# Autodesk Inventor assembly: 1103 Lift -Top Tier
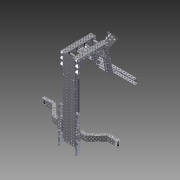
[picture p0: Inventor's stored thumbnail of the model, 180x180]
Saved by Autodesk Inventor 2012 (Build 160160000, 160)
## iProperties
Created: 2011-08-16
Part Number: 1103 Lift -Top Tier
Document SubType Name: Assembly
Designer: Dakota.Bayer
Author: Dakota.Bayer
## Documents named in this file (32)
- C:\Users\Wade\Documents\1103 Robot - CAD Assembly\1103 Lift -Top Tier.iam
- C:\Users\Wade\Documents\1103 Robot - CAD Assembly\5 x 30.ipt
- C:\Users\Wade\Documents\1103 Robot - CAD Assembly\1103 laddercustom1.ipt
- C:\Users\Wade\Documents\1103 Robot - CAD Assembly\2 x 12 c chan.ipt
- C:\Users\Wade\Documents\1103 Robot - CAD Assembly\1 x 10.ipt
- C:\Users\Wade\Documents\1103 Robot - CAD Assembly\Thin Black Spacer.ipt
- C:\Users\Wade\Documents\1103 Robot - CAD Assembly\2 x 20.ipt
- C:\Users\Wade\Documents\1103 Robot - CAD Assembly\2 x 41103 custom.ipt
- C:\Users\Wade\Documents\1103 Robot - CAD Assembly\2 x 15 custom!!!.iam
- C:\Users\Wade\Documents\1103 Robot - CAD Assembly\VEX-HINGE-PIN.ipt
- C:\Users\Wade\Documents\1103 Robot - CAD Assembly\VEX-HINGE-1 RevA.ipt
- C:\Users\Wade\Documents\24C VEX CAD Files\Standoffs & Couplers\Standoff 0.50''.ipt
- C:\Users\Wade\Documents\24C VEX CAD Files\Screws & Nuts\Screw 8-32 x 0.250''-Silver.ipt
- C:\Users\Wade\Documents\24C VEX CAD Files\Washers & Spacers\Spacer (Nylon), 0.375''.ipt
- C:\Users\Wade\Documents\24C VEX CAD Files\Screws & Nuts\Screw 8-32 x 0.750''-Silver.ipt
- C:\Users\Wade\Documents\24C VEX CAD Files\Screws & Nuts\Screw 8-32 x 0.375''-Silver.ipt
- C:\Users\Wade\Documents\24C VEX CAD Files\Screws & Nuts\Nut 8-32 Nylock.ipt
- C:\Users\Wade\Documents\24C VEX CAD Files\Washers & Spacers\Spacer (Nylon), 0.250''.ipt
- C:\Users\Wade\Documents\24C VEX CAD Files\Screws & Nuts\Screw 8-32 x 0.500''-Silver.ipt
- C:\Users\Wade\Documents\24C VEX CAD Files\Standoffs & Couplers\Standoff 0.75''.ipt
- C:\Users\Wade\Documents\24C VEX CAD Files\Standoffs & Couplers\Standoff 1.50''.ipt
- C:\Users\Wade\Documents\24C VEX CAD Files\Metal Other\Linear Slide Assembly-Parts\Linear Slide-Inner.ipt
- C:\Users\Wade\Documents\24C VEX CAD Files\Washers & Spacers\Spacer (Nylon), 0.4375''.ipt
- C:\Users\Wade\Documents\24C VEX CAD Files\Standoffs & Couplers\Standoff 3.00''.ipt
- C:\Users\Wade\Documents\24C VEX CAD Files\Standoffs & Couplers\Standoff 1.00''.ipt
- C:\Users\Wade\Documents\1103 Robot - CAD Assembly\.375'' Screw & Nylock Nut (Custom).iam
- C:\Users\Wade\Documents\1103 Robot - CAD Assembly\.375'' Screw & Nylock Nut.iam
- C:\Users\Wade\Documents\24C VEX CAD Files\Screws & Nuts\Screw 8-32 x 0.875''-Silver.ipt
- C:\Users\Wade\Documents\24C VEX CAD Files\Chain & Tank Tread\High Strength Chain Link.ipt
- C:\Users\Wade\Documents\1103 Robot - CAD Assembly\Ladder Mech.iam
- C:\Users\Wade\Documents\24C VEX CAD Files\Screws & Nuts\Screw 8-32 x 0.625''-Silver.ipt
- C:\Users\Wade\Documents\24C VEX CAD Files\Screws & Nuts\Screw 8-32 x 1.250''-Silver.ipt
## Components (161 placed, 31 different names)
1. 5 x 30:1 — Flush:33, Flush:34, Mate:310, Flush:35, Flush:36, Mate:328, Mate:693, Flush:43, Flush:44, Mate:757, Flush:53, Flush:54, Mate:774, Mate:775, Mate:776, Mate:778, Mate:779, Mate:780, Mate:823, Mate:825
2. Linear Slide-Inner:1
3. Standoff 0.50'':1
4. Screw 8-32 x 0.250''-Silver:1
5. Screw 8-32 x 0.250''-Silver:2
6. Screw 8-32 x 0.250''-Silver:3
7. Screw 8-32 x 0.250''-Silver:4
8. Standoff 0.50'':2
9. Screw 8-32 x 0.250''-Silver:5
10. Standoff 0.50'':3
11. Linear Slide-Inner:2
12. Screw 8-32 x 0.250''-Silver:6
13. Screw 8-32 x 0.250''-Silver:7
14. Screw 8-32 x 0.250''-Silver:8
15. Standoff 0.50'':4
16. Screw 8-32 x 0.250''-Silver:9 — Mate:804, Mate:805
17. 1103 laddercustom1:1 — Flush:33, Flush:34, Mate:474, Mate:818, Mate:819, Mate:821
18. Nut 8-32 Nylock:1
19. Nut 8-32 Nylock:2
20. Nut 8-32 Nylock:3
21. Screw 8-32 x 0.750''-Silver:4
22. Screw 8-32 x 0.750''-Silver:6 — Mate:818
23. Screw 8-32 x 0.750''-Silver:5 — Mate:820
24. 2 x 12 c chan:1 — Mate:310, Mate:459, Mate:474, Mate:500, Mate:505, Mate:512, Mate:515, Mate:837, Tangent:458, Tangent:459, Mate:840, Tangent:460, Tangent:461, Mate:841
25. Screw 8-32 x 0.375''-Silver:1
26. Screw 8-32 x 0.375''-Silver:2
27. Nut 8-32 Nylock:4
28. Nut 8-32 Nylock:5
29. 1103 laddercustom1:2 — Flush:35, Flush:36, Mate:484
30. Screw 8-32 x 0.750''-Silver:1 — Mate:822
31. Nut 8-32 Nylock:6
32. Screw 8-32 x 0.750''-Silver:2 — Mate:824
33. Nut 8-32 Nylock:7
34. 2 x 12 c chan:2 — Mate:328, Mate:460, Mate:484, Mate:503, Mate:507, Mate:509, Mate:518, Tangent:450, Tangent:451, Mate:835, Tangent:454, Tangent:455, Mate:838, Tangent:456, Tangent:457, Mate:839, Angle:1
35. Nut 8-32 Nylock:8
36. Screw 8-32 x 0.750''-Silver:3
37. Screw 8-32 x 0.375''-Silver:3
38. Nut 8-32 Nylock:9
39. Screw 8-32 x 0.375''-Silver:4
40. Nut 8-32 Nylock:10
41. 2 x 12 c chan:3 — Flush:37, Flush:38, Mate:460, Mate:525, Mate:794, Mate:795, Mate:796, Mate:797, Mate:798, Mate:799, Mate:828, Mate:829, Tangent:462, Tangent:463, Mate:876, Mate:877, Mate:885
42. 2 x 12 c chan:4 — Flush:37, Flush:38, Mate:459, Mate:788, Mate:789, Mate:790, Mate:791, Mate:792, Mate:793, Mate:814, Mate:815, Mate:875, Mate:881, Mate:884
43. 1 x 10:1 — Mate:843, Mate:872, Mate:875
44. 1 x 10:2 — Mate:525, Tangent:452, Tangent:453, Mate:845, Tangent:468, Tangent:469
45. Standoff 1.00'':1
46. Screw 8-32 x 0.375''-Silver:5
47. Screw 8-32 x 0.375''-Silver:6
48. Screw 8-32 x 0.375''-Silver:7
49. Screw 8-32 x 0.375''-Silver:8
50. Standoff 1.00'':2
51. Screw 8-32 x 0.375''-Silver:9
52. Screw 8-32 x 0.375''-Silver:10
53. Standoff 1.00'':3
54. Screw 8-32 x 0.375''-Silver:11
55. Screw 8-32 x 0.375''-Silver:12
56. Standoff 1.00'':4
57. Spacer (Nylon), 0.375'':1
58. Spacer (Nylon), 0.4375'':1 — Mate:819
59. Spacer (Nylon), 0.375'':6
60. Thin Black Spacer:1 — Mate:500
61. Thin Black Spacer:2 — Mate:503
62. Thin Black Spacer:3 — Mate:505
63. Thin Black Spacer:4 — Mate:507
64. Thin Black Spacer:5 — Mate:512
65. Thin Black Spacer:6 — Mate:509
66. Thin Black Spacer:7 — Mate:518
67. Thin Black Spacer:8 — Mate:515
68. Screw 8-32 x 0.375''-Silver:13
69. Screw 8-32 x 0.375''-Silver:14
70. Standoff 1.50'':1
71. Screw 8-32 x 0.375''-Silver:15
72. Screw 8-32 x 0.375''-Silver:16
73. Standoff 1.50'':2
74. Screw 8-32 x 0.375''-Silver:17
75. Screw 8-32 x 0.375''-Silver:18
76. Standoff 1.50'':3
77. Screw 8-32 x 0.375''-Silver:19
78. Screw 8-32 x 0.375''-Silver:20
79. Standoff 1.50'':4
80. Screw 8-32 x 0.375''-Silver:21
81. Screw 8-32 x 0.375''-Silver:22
82. Standoff 1.50'':5
83. Standoff 3.00'':1
84. Spacer (Nylon), 0.250'':1 — Mate:873
85. Spacer (Nylon), 0.250'':2
86. Screw 8-32 x 0.500''-Silver:1
87. Screw 8-32 x 0.500''-Silver:2 — Mate:872
88. Screw 8-32 x 0.500''-Silver:3
89. Screw 8-32 x 0.500''-Silver:4
90. Spacer (Nylon), 0.250'':3 — Mate:874
91. Standoff 3.00'':2 — Mate:873, Mate:874
92. Spacer (Nylon), 0.250'':4
93. 2 x 20:1 — Mate:800, Mate:801, Mate:802, Mate:803, Mate:805, Mate:807, Mate:810, Mate:811
94. Screw 8-32 x 0.625''-Silver:2 — Mate:879, Mate:889, Mate:890
95. Screw 8-32 x 0.625''-Silver:1 — Mate:880, Mate:886, Mate:891
96. Standoff 0.50'':5 — Mate:765, Mate:768, Mate:854
97. Standoff 0.50'':6 — Mate:760, Mate:763, Mate:846, Mate:905
98. Standoff 0.50'':7 — Mate:766, Mate:767, Mate:856
99. Standoff 0.50'':8 — Mate:761, Mate:762, Mate:848
100. Standoff 0.50'':9 — Mate:773, Mate:777, Mate:778, Mate:779, Mate:780, Mate:860
101. Standoff 0.50'':10 — Mate:770, Mate:771, Mate:772, Mate:774, Mate:775, Mate:776, Mate:858
102. 2 x 41103 custom:1 — Mate:693, Flush:43, Flush:44, Flush:66, Flush:67, Mate:904
103. 2 x 15 custom!!!:1 [sub-assembly] — Flush:66, Flush:67, Mate:894, Mate:896, Mate:897, Mate:904
104. Standoff 0.50'':11 — Mate:783, Mate:784, Mate:850
105. Standoff 0.50'':12 — Mate:782, Mate:785, Mate:852
106. 2 x 15 custom!!!:2 [sub-assembly] — Flush:64, Flush:65, Mate:898, Mate:900, Mate:901, Mate:903
107. 2 x 41103 custom:2 — Mate:757, Flush:53, Flush:54, Flush:64, Flush:65, Mate:903
108. VEX-HINGE-PIN:1 — Mate:759, Flush:60
109. VEX-HINGE-1 RevA:1 — Mate:759, Flush:60, Mate:760, Mate:761, Mate:762, Mate:763, Mate:847, Mate:849, Mate:905
110. VEX-HINGE-1 RevA:2 — Mate:764, Flush:61, Mate:765, Mate:766, Mate:767, Mate:768, Mate:855, Mate:857
111. VEX-HINGE-PIN:2 — Mate:764, Flush:61
112. VEX-HINGE-1 RevA:3 — Mate:769, Flush:62, Mate:770, Mate:771, Mate:772, Mate:773, Mate:777, Mate:859, Mate:861
113. VEX-HINGE-PIN:3 — Mate:769, Flush:62
114. VEX-HINGE-1 RevA:4 — Flush:63, Mate:781, Mate:782, Mate:783, Mate:784, Mate:785, Mate:851, Mate:853
115. VEX-HINGE-PIN:4 — Flush:63, Mate:781
116. Standoff 0.75'':1 — Mate:788, Mate:789, Mate:790, Mate:804, Mate:813
117. Standoff 0.75'':2 — Mate:794, Mate:795, Mate:796, Mate:809, Mate:826
118. Standoff 0.75'':3 — Mate:797, Mate:798, Mate:799, Mate:800, Mate:801, Mate:802, Mate:808, Mate:827
119. Standoff 0.75'':4 — Mate:791, Mate:792, Mate:793, Mate:803, Mate:806, Mate:812
120. Screw 8-32 x 0.250''-Silver:10 — Mate:806, Mate:807
121. Screw 8-32 x 0.250''-Silver:11 — Mate:808, Mate:811
122. Screw 8-32 x 0.250''-Silver:12 — Mate:809, Mate:810
123. Screw 8-32 x 0.250''-Silver:13 — Mate:812, Mate:814
124. Screw 8-32 x 0.250''-Silver:14 — Mate:813, Mate:815
125. Spacer (Nylon), 0.4375'':2 — Mate:820, Mate:821
126. Spacer (Nylon), 0.4375'':3 — Mate:824, Mate:825
127. Spacer (Nylon), 0.4375'':4 — Mate:822, Mate:823
128. Screw 8-32 x 0.250''-Silver:15 — Mate:827, Mate:829
129. Screw 8-32 x 0.250''-Silver:16 — Mate:826, Mate:828
130. .375'' Screw & Nylock Nut (Custom):1 [sub-assembly] — Tangent:450, Tangent:451, Mate:835, Tangent:452, Tangent:453, Mate:836
131. .375'' Screw & Nylock Nut (Custom):2 [sub-assembly] — Mate:836, Mate:837
132. .375'' Screw & Nylock Nut:1 [sub-assembly] — Tangent:454, Tangent:455, Mate:838, Tangent:462, Tangent:463
133. .375'' Screw & Nylock Nut:2 [sub-assembly] — Tangent:460, Tangent:461, Mate:841
134. .375'' Screw & Nylock Nut:3 [sub-assembly] — Tangent:458, Tangent:459, Mate:840
135. .375'' Screw & Nylock Nut:4 [sub-assembly] — Tangent:456, Tangent:457, Mate:839
136. .375'' Screw & Nylock Nut:5 [sub-assembly] — Mate:843, Mate:878
137. .375'' Screw & Nylock Nut:6 [sub-assembly] — Mate:845, Mate:876, Mate:877, Tangent:468, Tangent:469, Mate:878
138. Screw 8-32 x 0.250''-Silver:17 — Mate:848, Mate:849
139. Screw 8-32 x 0.250''-Silver:18 — Mate:850, Mate:851
140. Screw 8-32 x 0.250''-Silver:19 — Mate:852, Mate:853
141. Screw 8-32 x 0.250''-Silver:20 — Mate:846, Mate:847
142. Screw 8-32 x 0.250''-Silver:21 — Mate:854, Mate:855
143. Screw 8-32 x 0.250''-Silver:22 — Mate:856, Mate:857
144. Screw 8-32 x 0.250''-Silver:23 — Mate:858, Mate:859
145. Screw 8-32 x 0.250''-Silver:24 — Mate:860, Mate:861
146. Screw 8-32 x 0.875''-Silver:1 — Mate:865, Tangent:466, Tangent:467
147. Nut 8-32 Nylock:21 — Mate:865, Mate:869
148. Spacer (Nylon), 0.375'':7 — Mate:868, Mate:869, Mate:870
149. High Strength Chain Link:1 — Mate:868, Tangent:466, Mate:870, Tangent:467, Mate:871, Flush:68
150. High Strength Chain Link:2 — Mate:871, Flush:68
151. Ladder Mech:1 [sub-assembly] — Mate:879, Mate:880, Mate:881, Mate:882, Mate:883, Angle:1
152. Screw 8-32 x 0.750''-Silver:7 — Mate:882, Mate:885, Mate:887, Mate:892
153. Screw 8-32 x 0.750''-Silver:8 — Mate:883, Mate:884, Mate:888, Mate:893
154. Nut 8-32 Nylock:22 — Mate:888, Mate:893
155. Nut 8-32 Nylock:23 — Mate:889, Mate:890
156. Nut 8-32 Nylock:24 — Mate:887, Mate:892
157. Nut 8-32 Nylock:25 — Mate:886, Mate:891
158. Nut 8-32 Nylock:26 — Mate:895, Mate:896
159. Screw 8-32 x 1.250''-Silver:1 — Mate:894, Mate:895, Mate:897
160. Nut 8-32 Nylock:27 — Mate:900, Mate:902
161. Screw 8-32 x 1.250''-Silver:2 — Mate:898, Mate:901, Mate:902
## Relationships (415: Mate 274, Tangent 120, Flush 20, Angle 1)
- [Flush]: 5 x 30:1 ↔ Linear Slide-Inner:1
- [Mate]: 5 x 30:1 ↔ Standoff 0.50'':1
- [Mate]: 5 x 30:1 ↔ Screw 8-32 x 0.250''-Silver:1
- [Mate]: Linear Slide-Inner:1 ↔ Screw 8-32 x 0.250''-Silver:2
- [Mate]: Standoff 0.50'':1 ↔ Screw 8-32 x 0.250''-Silver:1
- [Mate]: Standoff 0.50'':1 ↔ Screw 8-32 x 0.250''-Silver:2
- [Mate]: Linear Slide-Inner:1 ↔ Standoff 0.50'':1
- [Mate]: Linear Slide-Inner:1 ↔ Screw 8-32 x 0.250''-Silver:4
- [Tangent] (0.2286 mm): Linear Slide-Inner:1 ↔ Screw 8-32 x 0.250''-Silver:4
- [Tangent] (0.2286 mm): Linear Slide-Inner:1 ↔ Screw 8-32 x 0.250''-Silver:4
- [Mate]: Linear Slide-Inner:1 ↔ Standoff 0.50'':2
- [Mate]: Screw 8-32 x 0.250''-Silver:4 ↔ Standoff 0.50'':2
- [Mate]: 5 x 30:1 ↔ Standoff 0.50'':2
- [Mate]: 5 x 30:1 ↔ Screw 8-32 x 0.250''-Silver:3
- [Mate]: 5 x 30:1 ↔ Screw 8-32 x 0.250''-Silver:5
- [Mate]: 5 x 30:1 ↔ Standoff 0.50'':3
- [Mate]: Screw 8-32 x 0.250''-Silver:5 ↔ Standoff 0.50'':3
- [Mate]: Standoff 0.50'':3 ↔ Linear Slide-Inner:2
- [Mate]: Linear Slide-Inner:2 ↔ Screw 8-32 x 0.250''-Silver:6
- [Tangent] (0.2286 mm): Linear Slide-Inner:2 ↔ Screw 8-32 x 0.250''-Silver:6
- [Tangent] (0.2286 mm): Linear Slide-Inner:2 ↔ Screw 8-32 x 0.250''-Silver:6
- [Mate]: Standoff 0.50'':3 ↔ Screw 8-32 x 0.250''-Silver:6
- [Mate]: 5 x 30:1 ↔ Screw 8-32 x 0.250''-Silver:7
- [Tangent] (0.2286 mm): 5 x 30:1 ↔ Screw 8-32 x 0.250''-Silver:7
- [Tangent] (0.2286 mm): 5 x 30:1 ↔ Screw 8-32 x 0.250''-Silver:7
- [Mate]: Linear Slide-Inner:2 ↔ Screw 8-32 x 0.250''-Silver:8
- [Mate]: 5 x 30:1 ↔ Standoff 0.50'':4
- [Mate]: Linear Slide-Inner:2 ↔ Standoff 0.50'':4
- [Mate]: Screw 8-32 x 0.250''-Silver:8 ↔ Standoff 0.50'':4
- [Mate]: Screw 8-32 x 0.250''-Silver:7 ↔ Standoff 0.50'':4
- Flush:33: 5 x 30:1 ↔ 1103 laddercustom1:1
- Flush:34: 5 x 30:1 ↔ 1103 laddercustom1:1
- [Mate]: 5 x 30:1 ↔ Nut 8-32 Nylock:1
- [Mate]: 5 x 30:1 ↔ Nut 8-32 Nylock:2
- [Mate]: 5 x 30:1 ↔ Nut 8-32 Nylock:3
- [Tangent] (0.2286 mm): 1103 laddercustom1:1 ↔ Screw 8-32 x 0.750''-Silver:6
- [Tangent] (0.2286 mm): 1103 laddercustom1:1 ↔ Screw 8-32 x 0.750''-Silver:6
- [Mate]: Nut 8-32 Nylock:3 ↔ Screw 8-32 x 0.750''-Silver:6
- [Tangent] (0.2286 mm): 1103 laddercustom1:1 ↔ Screw 8-32 x 0.750''-Silver:5
- [Tangent] (0.2286 mm): 1103 laddercustom1:1 ↔ Screw 8-32 x 0.750''-Silver:5
- [Mate]: Nut 8-32 Nylock:2 ↔ Screw 8-32 x 0.750''-Silver:5
- [Tangent] (0.2286 mm): 1103 laddercustom1:1 ↔ Screw 8-32 x 0.750''-Silver:4
- [Tangent] (0.2286 mm): 1103 laddercustom1:1 ↔ Screw 8-32 x 0.750''-Silver:4
- [Tangent] (0.2286 mm): Screw 8-32 x 0.750''-Silver:4 ↔ 2 x 12 c chan:1
- Mate:310: 5 x 30:1 ↔ 2 x 12 c chan:1
- [Tangent] (0.2286 mm): Screw 8-32 x 0.750''-Silver:4 ↔ 2 x 12 c chan:1
- [Tangent] (0.2286 mm): 1103 laddercustom1:1 ↔ Screw 8-32 x 0.375''-Silver:1
- [Tangent] (0.2286 mm): 1103 laddercustom1:1 ↔ Screw 8-32 x 0.375''-Silver:1
- [Tangent] (0.2286 mm): 1103 laddercustom1:1 ↔ Screw 8-32 x 0.375''-Silver:2
- [Tangent] (0.2286 mm): 1103 laddercustom1:1 ↔ Screw 8-32 x 0.375''-Silver:2
- [Mate]: Screw 8-32 x 0.375''-Silver:2 ↔ Nut 8-32 Nylock:5
- [Mate]: Screw 8-32 x 0.375''-Silver:1 ↔ Nut 8-32 Nylock:4
- Flush:35: 5 x 30:1 ↔ 1103 laddercustom1:2
- Flush:36: 5 x 30:1 ↔ 1103 laddercustom1:2
- [Tangent] (0.2286 mm): 1103 laddercustom1:2 ↔ Screw 8-32 x 0.750''-Silver:1
- [Tangent] (0.2286 mm): 1103 laddercustom1:2 ↔ Screw 8-32 x 0.750''-Silver:1
- [Mate]: 5 x 30:1 ↔ Nut 8-32 Nylock:6
- [Mate]: Screw 8-32 x 0.750''-Silver:1 ↔ Nut 8-32 Nylock:6
- [Tangent] (0.2286 mm): 1103 laddercustom1:2 ↔ Screw 8-32 x 0.750''-Silver:2
- [Tangent] (0.2286 mm): 1103 laddercustom1:2 ↔ Screw 8-32 x 0.750''-Silver:2
- [Mate]: 5 x 30:1 ↔ Nut 8-32 Nylock:7
- [Mate]: Screw 8-32 x 0.750''-Silver:2 ↔ Nut 8-32 Nylock:7
- Mate:328: 5 x 30:1 ↔ 2 x 12 c chan:2
- [Tangent] (0.2286 mm): 1103 laddercustom1:2 ↔ Screw 8-32 x 0.750''-Silver:3
- [Tangent] (0.2286 mm): 1103 laddercustom1:2 ↔ Screw 8-32 x 0.750''-Silver:3
- [Tangent] (0.2286 mm): 5 x 30:1 ↔ Screw 8-32 x 0.750''-Silver:3
- [Tangent] (0.2286 mm): 5 x 30:1 ↔ Screw 8-32 x 0.750''-Silver:3
- [Mate]: 5 x 30:1 ↔ Nut 8-32 Nylock:8
- [Mate]: Nut 8-32 Nylock:8 ↔ Screw 8-32 x 0.750''-Silver:3
- [Tangent] (0.2286 mm): 1103 laddercustom1:2 ↔ Screw 8-32 x 0.375''-Silver:3
- [Tangent] (0.2286 mm): 1103 laddercustom1:2 ↔ Screw 8-32 x 0.375''-Silver:3
- [Mate]: Screw 8-32 x 0.375''-Silver:3 ↔ Nut 8-32 Nylock:9
- [Tangent] (0.2286 mm): 1103 laddercustom1:2 ↔ Screw 8-32 x 0.375''-Silver:4
- [Tangent] (0.2286 mm): 1103 laddercustom1:2 ↔ Screw 8-32 x 0.375''-Silver:4
- [Mate]: Screw 8-32 x 0.375''-Silver:4 ↔ Nut 8-32 Nylock:10
- [Tangent] (0.2286 mm): 2 x 12 c chan:2 ↔ Screw 8-32 x 0.750''-Silver:3
- [Mate]: 2 x 12 c chan:1 ↔ Screw 8-32 x 0.375''-Silver:6
- [Tangent] (0.2286 mm): 2 x 12 c chan:1 ↔ Screw 8-32 x 0.375''-Silver:6
- [Tangent] (0.2286 mm): 2 x 12 c chan:1 ↔ Screw 8-32 x 0.375''-Silver:6
- [Mate]: 2 x 12 c chan:2 ↔ Screw 8-32 x 0.375''-Silver:5
- [Tangent] (0.2286 mm): 2 x 12 c chan:2 ↔ Screw 8-32 x 0.375''-Silver:5
- [Tangent] (0.2286 mm): 2 x 12 c chan:2 ↔ Screw 8-32 x 0.375''-Silver:5
- [Mate]: Standoff 1.00'':1 ↔ Screw 8-32 x 0.375''-Silver:5
- [Mate]: 2 x 12 c chan:1 ↔ Screw 8-32 x 0.375''-Silver:7
- [Tangent] (0.2286 mm): 2 x 12 c chan:1 ↔ Screw 8-32 x 0.375''-Silver:7
- [Tangent] (0.2286 mm): 2 x 12 c chan:1 ↔ Screw 8-32 x 0.375''-Silver:7
- [Mate]: 2 x 12 c chan:2 ↔ Screw 8-32 x 0.375''-Silver:8
- [Tangent] (0.2286 mm): 2 x 12 c chan:2 ↔ Screw 8-32 x 0.375''-Silver:8
- [Tangent] (0.2286 mm): 2 x 12 c chan:2 ↔ Screw 8-32 x 0.375''-Silver:8
- [Mate]: Screw 8-32 x 0.375''-Silver:8 ↔ Standoff 1.00'':2
- [Mate]: 2 x 12 c chan:1 ↔ Screw 8-32 x 0.375''-Silver:9
- [Tangent] (0.2286 mm): 2 x 12 c chan:1 ↔ Screw 8-32 x 0.375''-Silver:9
- [Tangent] (0.2286 mm): 2 x 12 c chan:1 ↔ Screw 8-32 x 0.375''-Silver:9
- [Mate]: 2 x 12 c chan:2 ↔ Screw 8-32 x 0.375''-Silver:10
- [Tangent] (0.2286 mm): 2 x 12 c chan:2 ↔ Screw 8-32 x 0.375''-Silver:10
- [Tangent] (0.2286 mm): 2 x 12 c chan:2 ↔ Screw 8-32 x 0.375''-Silver:10
- [Mate]: Screw 8-32 x 0.375''-Silver:9 ↔ Standoff 1.00'':3
- [Mate]: 2 x 12 c chan:2 ↔ Screw 8-32 x 0.375''-Silver:12
- [Tangent] (0.2286 mm): 2 x 12 c chan:2 ↔ Screw 8-32 x 0.375''-Silver:12
- [Tangent] (0.2286 mm): 2 x 12 c chan:2 ↔ Screw 8-32 x 0.375''-Silver:12
- [Mate]: 2 x 12 c chan:1 ↔ Screw 8-32 x 0.375''-Silver:11
- [Tangent] (0.2286 mm): 2 x 12 c chan:1 ↔ Screw 8-32 x 0.375''-Silver:11
- [Tangent] (0.2286 mm): 2 x 12 c chan:1 ↔ Screw 8-32 x 0.375''-Silver:11
- [Mate]: Screw 8-32 x 0.375''-Silver:12 ↔ Standoff 1.00'':4
- Flush:37: 2 x 12 c chan:3 ↔ 2 x 12 c chan:4
- Flush:38: 2 x 12 c chan:3 ↔ 2 x 12 c chan:4
- Mate:459: 2 x 12 c chan:1 ↔ 2 x 12 c chan:4
- Mate:460: 2 x 12 c chan:2 ↔ 2 x 12 c chan:3
- [Mate]: 5 x 30:1 ↔ Spacer (Nylon), 0.375'':1
- [Mate]: Screw 8-32 x 0.750''-Silver:4 ↔ Spacer (Nylon), 0.375'':1
- Mate:474: 1103 laddercustom1:1 ↔ 2 x 12 c chan:1
- [Mate]: 2 x 12 c chan:1 ↔ Spacer (Nylon), 0.375'':1
- [Mate]: 1103 laddercustom1:1 ↔ Screw 8-32 x 0.750''-Silver:4
- [Mate]: 1103 laddercustom1:1 ↔ Screw 8-32 x 0.375''-Silver:1
- [Mate]: 1103 laddercustom1:1 ↔ Screw 8-32 x 0.375''-Silver:2
- [Mate]: 1103 laddercustom1:1 ↔ Screw 8-32 x 0.750''-Silver:5
- [Mate]: Screw 8-32 x 0.750''-Silver:6 ↔ Spacer (Nylon), 0.4375'':1
- Mate:484: 1103 laddercustom1:2 ↔ 2 x 12 c chan:2
- [Mate]: 1103 laddercustom1:2 ↔ Screw 8-32 x 0.750''-Silver:3
- [Mate]: 5 x 30:1 ↔ Spacer (Nylon), 0.375'':6
- [Mate]: 2 x 12 c chan:2 ↔ Spacer (Nylon), 0.375'':6
- [Mate]: Screw 8-32 x 0.750''-Silver:3 ↔ Spacer (Nylon), 0.375'':6
- [Mate]: 1103 laddercustom1:2 ↔ Screw 8-32 x 0.750''-Silver:2
- [Mate]: 1103 laddercustom1:2 ↔ Screw 8-32 x 0.750''-Silver:1
- [Mate]: 2 x 12 c chan:2 ↔ Nut 8-32 Nylock:10
- [Mate]: 2 x 12 c chan:2 ↔ Nut 8-32 Nylock:9
- [Mate]: Nut 8-32 Nylock:1 ↔ Screw 8-32 x 0.750''-Silver:4
- Mate:500: 2 x 12 c chan:1 ↔ Thin Black Spacer:1
- [Mate]: Screw 8-32 x 0.375''-Silver:11 ↔ Thin Black Spacer:1
- [Mate]: Standoff 1.00'':4 ↔ Thin Black Spacer:1
- Mate:503: 2 x 12 c chan:2 ↔ Thin Black Spacer:2
- [Mate]: Screw 8-32 x 0.375''-Silver:12 ↔ Thin Black Spacer:2
- Mate:505: 2 x 12 c chan:1 ↔ Thin Black Spacer:3
- [Mate]: Screw 8-32 x 0.375''-Silver:9 ↔ Thin Black Spacer:3
- Mate:507: 2 x 12 c chan:2 ↔ Thin Black Spacer:4
- [Mate]: Screw 8-32 x 0.375''-Silver:10 ↔ Thin Black Spacer:4
- Mate:509: 2 x 12 c chan:2 ↔ Thin Black Spacer:6
- [Mate]: Screw 8-32 x 0.375''-Silver:8 ↔ Thin Black Spacer:6
- [Mate]: Standoff 1.00'':3 ↔ Thin Black Spacer:3
- Mate:512: 2 x 12 c chan:1 ↔ Thin Black Spacer:5
- [Mate]: Screw 8-32 x 0.375''-Silver:7 ↔ Thin Black Spacer:5
- [Mate]: Standoff 1.00'':2 ↔ Thin Black Spacer:5
- Mate:515: 2 x 12 c chan:1 ↔ Thin Black Spacer:8
- [Mate]: Screw 8-32 x 0.375''-Silver:6 ↔ Thin Black Spacer:8
- [Mate]: Standoff 1.00'':1 ↔ Thin Black Spacer:8
- Mate:518: 2 x 12 c chan:2 ↔ Thin Black Spacer:7
- [Mate]: Screw 8-32 x 0.375''-Silver:5 ↔ Thin Black Spacer:7
- Mate:525: 2 x 12 c chan:3 ↔ 1 x 10:2
- [Tangent] (0.2286 mm): 2 x 12 c chan:4 ↔ Screw 8-32 x 0.375''-Silver:13
- [Tangent] (0.2286 mm): 2 x 12 c chan:4 ↔ Screw 8-32 x 0.375''-Silver:13
- [Mate]: 2 x 12 c chan:3 ↔ Screw 8-32 x 0.375''-Silver:14
- [Tangent] (0.2286 mm): 2 x 12 c chan:3 ↔ Screw 8-32 x 0.375''-Silver:14
- [Tangent] (0.2286 mm): 2 x 12 c chan:3 ↔ Screw 8-32 x 0.375''-Silver:14
- [Mate]: 2 x 12 c chan:4 ↔ Screw 8-32 x 0.375''-Silver:13
- [Mate]: 2 x 12 c chan:3 ↔ Standoff 1.50'':1
- [Mate]: Screw 8-32 x 0.375''-Silver:14 ↔ Standoff 1.50'':1
- [Mate]: 2 x 12 c chan:3 ↔ Screw 8-32 x 0.375''-Silver:17
- [Tangent] (0.2286 mm): 2 x 12 c chan:3 ↔ Screw 8-32 x 0.375''-Silver:17
- [Tangent] (0.2286 mm): 2 x 12 c chan:3 ↔ Screw 8-32 x 0.375''-Silver:17
- [Mate]: 2 x 12 c chan:4 ↔ Screw 8-32 x 0.375''-Silver:15
- [Tangent] (0.2286 mm): 2 x 12 c chan:4 ↔ Screw 8-32 x 0.375''-Silver:15
- [Tangent] (0.2286 mm): 2 x 12 c chan:4 ↔ Screw 8-32 x 0.375''-Silver:15
- [Mate]: 2 x 12 c chan:3 ↔ Standoff 1.50'':2
- [Mate]: Standoff 1.50'':2 ↔ Screw 8-32 x 0.375''-Silver:17
- [Mate]: 2 x 12 c chan:4 ↔ Screw 8-32 x 0.375''-Silver:18
- [Tangent] (0.2286 mm): 2 x 12 c chan:4 ↔ Screw 8-32 x 0.375''-Silver:18
- [Tangent] (0.2286 mm): 2 x 12 c chan:4 ↔ Screw 8-32 x 0.375''-Silver:18
- [Mate]: 2 x 12 c chan:3 ↔ Screw 8-32 x 0.375''-Silver:16
- [Tangent] (0.2286 mm): 2 x 12 c chan:3 ↔ Screw 8-32 x 0.375''-Silver:16
- [Tangent] (0.2286 mm): 2 x 12 c chan:3 ↔ Screw 8-32 x 0.375''-Silver:16
- [Mate]: 2 x 12 c chan:3 ↔ Standoff 1.50'':3
- [Mate]: Screw 8-32 x 0.375''-Silver:16 ↔ Standoff 1.50'':3
- [Mate]: 2 x 12 c chan:4 ↔ Screw 8-32 x 0.375''-Silver:19
- [Tangent] (0.2286 mm): 2 x 12 c chan:4 ↔ Screw 8-32 x 0.375''-Silver:19
- [Tangent] (0.2286 mm): 2 x 12 c chan:4 ↔ Screw 8-32 x 0.375''-Silver:19
- [Mate]: 2 x 12 c chan:3 ↔ Screw 8-32 x 0.375''-Silver:20
- [Tangent] (0.2286 mm): 2 x 12 c chan:3 ↔ Screw 8-32 x 0.375''-Silver:20
- [Tangent] (0.2286 mm): 2 x 12 c chan:3 ↔ Screw 8-32 x 0.375''-Silver:20
- [Mate]: 2 x 12 c chan:3 ↔ Standoff 1.50'':4
- [Mate]: Screw 8-32 x 0.375''-Silver:20 ↔ Standoff 1.50'':4
- [Mate]: 2 x 12 c chan:4 ↔ Screw 8-32 x 0.375''-Silver:21
- [Tangent] (0.2286 mm): 2 x 12 c chan:4 ↔ Screw 8-32 x 0.375''-Silver:21
- [Tangent] (0.2286 mm): 2 x 12 c chan:4 ↔ Screw 8-32 x 0.375''-Silver:21
- [Mate]: 2 x 12 c chan:3 ↔ Screw 8-32 x 0.375''-Silver:22
- [Tangent] (0.2286 mm): 2 x 12 c chan:3 ↔ Screw 8-32 x 0.375''-Silver:22
- [Tangent] (0.2286 mm): 2 x 12 c chan:3 ↔ Screw 8-32 x 0.375''-Silver:22
- [Mate]: 2 x 12 c chan:3 ↔ Standoff 1.50'':5
- [Mate]: Screw 8-32 x 0.375''-Silver:22 ↔ Standoff 1.50'':5
- [Mate]: 1 x 10:2 ↔ Screw 8-32 x 0.500''-Silver:1
- [Tangent] (0.2286 mm): 1 x 10:2 ↔ Screw 8-32 x 0.500''-Silver:1
- [Tangent] (0.2286 mm): 1 x 10:2 ↔ Screw 8-32 x 0.500''-Silver:1
- [Tangent] (0.2286 mm): 1 x 10:1 ↔ Screw 8-32 x 0.500''-Silver:2
- [Tangent] (0.2286 mm): 1 x 10:1 ↔ Screw 8-32 x 0.500''-Silver:2
- [Mate]: Spacer (Nylon), 0.250'':1 ↔ Screw 8-32 x 0.500''-Silver:2
- [Mate]: 1 x 10:2 ↔ Spacer (Nylon), 0.250'':2
- [Mate]: Spacer (Nylon), 0.250'':2 ↔ Screw 8-32 x 0.500''-Silver:1
- [Mate]: Standoff 3.00'':1 ↔ Spacer (Nylon), 0.250'':2
- [Mate]: Standoff 3.00'':1 ↔ Spacer (Nylon), 0.250'':1
- [Mate]: 1 x 10:2 ↔ Screw 8-32 x 0.500''-Silver:3
- [Tangent] (0.2286 mm): 1 x 10:2 ↔ Screw 8-32 x 0.500''-Silver:3
- [Tangent] (0.2286 mm): 1 x 10:2 ↔ Screw 8-32 x 0.500''-Silver:3
- [Mate]: 1 x 10:1 ↔ Screw 8-32 x 0.500''-Silver:4
- [Tangent] (0.2286 mm): 1 x 10:1 ↔ Screw 8-32 x 0.500''-Silver:4
- [Tangent] (0.2286 mm): 1 x 10:1 ↔ Screw 8-32 x 0.500''-Silver:4
- [Mate]: Screw 8-32 x 0.500''-Silver:4 ↔ Spacer (Nylon), 0.250'':3
- [Mate]: 1 x 10:2 ↔ Spacer (Nylon), 0.250'':4
- [Mate]: Screw 8-32 x 0.500''-Silver:3 ↔ Spacer (Nylon), 0.250'':4
- [Mate]: Standoff 3.00'':2 ↔ Spacer (Nylon), 0.250'':4
- [Mate]: Screw 8-32 x 0.500''-Silver:3 ↔ Standoff 3.00'':2
- [Mate]: 2 x 12 c chan:4 ↔ Screw 8-32 x 0.625''-Silver:2
- [Tangent] (0.2286 mm): 2 x 12 c chan:4 ↔ Screw 8-32 x 0.625''-Silver:2
- [Tangent] (0.2286 mm): 2 x 12 c chan:4 ↔ Screw 8-32 x 0.625''-Silver:2
- [Mate]: 2 x 12 c chan:3 ↔ Screw 8-32 x 0.625''-Silver:1
- [Tangent] (0.2286 mm): 2 x 12 c chan:3 ↔ Screw 8-32 x 0.625''-Silver:1
- [Tangent] (0.2286 mm): 2 x 12 c chan:3 ↔ Screw 8-32 x 0.625''-Silver:1
- [Tangent] (0.2286 mm): Linear Slide-Inner:2 ↔ Screw 8-32 x 0.250''-Silver:8
- [Tangent] (0.2286 mm): Linear Slide-Inner:2 ↔ Screw 8-32 x 0.250''-Silver:8
- [Tangent] (0.2286 mm): 5 x 30:1 ↔ Screw 8-32 x 0.250''-Silver:5
- [Tangent] (0.2286 mm): 5 x 30:1 ↔ Screw 8-32 x 0.250''-Silver:5
- [Tangent] (0.2286 mm): Linear Slide-Inner:1 ↔ Screw 8-32 x 0.250''-Silver:2
- [Tangent] (0.2286 mm): Linear Slide-Inner:1 ↔ Screw 8-32 x 0.250''-Silver:2
- [Tangent] (0.2286 mm): 5 x 30:1 ↔ Screw 8-32 x 0.250''-Silver:1
- [Tangent] (0.2286 mm): 5 x 30:1 ↔ Screw 8-32 x 0.250''-Silver:1
- [Tangent] (0.2286 mm): 5 x 30:1 ↔ Screw 8-32 x 0.250''-Silver:3
- [Tangent] (0.2286 mm): 5 x 30:1 ↔ Screw 8-32 x 0.250''-Silver:3
- [Mate]: 5 x 30:1 ↔ Standoff 0.50'':5
- [Tangent] (0.2286 mm): 5 x 30:1 ↔ Standoff 0.50'':5
- [Tangent] (0.2286 mm): 5 x 30:1 ↔ Standoff 0.50'':5
- [Mate]: 5 x 30:1 ↔ Standoff 0.50'':6
- [Tangent] (0.2159 mm): 5 x 30:1 ↔ Standoff 0.50'':6
- [Tangent] (0.2159 mm): 5 x 30:1 ↔ Standoff 0.50'':6
- [Mate]: 5 x 30:1 ↔ Standoff 0.50'':7
- [Tangent] (0.2286 mm): 5 x 30:1 ↔ Standoff 0.50'':5
- [Tangent] (0.2286 mm): 5 x 30:1 ↔ Standoff 0.50'':7
- [Tangent] (0.2286 mm): 5 x 30:1 ↔ Standoff 0.50'':7
- [Mate]: 5 x 30:1 ↔ Standoff 0.50'':8
- [Tangent] (0.2159 mm): 5 x 30:1 ↔ Standoff 0.50'':8
- [Tangent] (0.2159 mm): 5 x 30:1 ↔ Standoff 0.50'':8
- Mate:693: 5 x 30:1 ↔ 2 x 41103 custom:1
- Flush:43: 5 x 30:1 ↔ 2 x 41103 custom:1
- Flush:44: 5 x 30:1 ↔ 2 x 41103 custom:1
- [Mate]: 5 x 30:1 ↔ Standoff 0.50'':11
- [Mate]: 5 x 30:1 ↔ Standoff 0.50'':12
- [Tangent] (0.2286 mm): 5 x 30:1 ↔ Standoff 0.50'':12
- [Tangent] (0.2286 mm): 5 x 30:1 ↔ Standoff 0.50'':12
- [Tangent] (0.2286 mm): 5 x 30:1 ↔ Standoff 0.50'':11
- [Tangent] (0.2286 mm): 5 x 30:1 ↔ Standoff 0.50'':11
- Mate:757: 5 x 30:1 ↔ 2 x 41103 custom:2
- Flush:53: 5 x 30:1 ↔ 2 x 41103 custom:2
- Flush:54: 5 x 30:1 ↔ 2 x 41103 custom:2
- Mate:759: VEX-HINGE-PIN:1 ↔ VEX-HINGE-1 RevA:1
- Flush:60: VEX-HINGE-PIN:1 ↔ VEX-HINGE-1 RevA:1
- Mate:760: Standoff 0.50'':6 ↔ VEX-HINGE-1 RevA:1
- Mate:761 (2.3114 mm): Standoff 0.50'':8 ↔ VEX-HINGE-1 RevA:1
- Mate:762 (2.3114 mm): Standoff 0.50'':8 ↔ VEX-HINGE-1 RevA:1
- Mate:763 (2.3114 mm): Standoff 0.50'':6 ↔ VEX-HINGE-1 RevA:1
- Mate:764: VEX-HINGE-1 RevA:2 ↔ VEX-HINGE-PIN:2
- Flush:61: VEX-HINGE-1 RevA:2 ↔ VEX-HINGE-PIN:2
- Mate:765: Standoff 0.50'':5 ↔ VEX-HINGE-1 RevA:2
- Mate:766 (2.3114 mm): Standoff 0.50'':7 ↔ VEX-HINGE-1 RevA:2
- Mate:767 (2.3114 mm): Standoff 0.50'':7 ↔ VEX-HINGE-1 RevA:2
- Mate:768 (2.3114 mm): Standoff 0.50'':5 ↔ VEX-HINGE-1 RevA:2
- Mate:769: VEX-HINGE-1 RevA:3 ↔ VEX-HINGE-PIN:3
- Flush:62: VEX-HINGE-1 RevA:3 ↔ VEX-HINGE-PIN:3
- Mate:770: Standoff 0.50'':10 ↔ VEX-HINGE-1 RevA:3
- Mate:771 (2.3114 mm): Standoff 0.50'':10 ↔ VEX-HINGE-1 RevA:3
- Mate:772 (2.3114 mm): Standoff 0.50'':10 ↔ VEX-HINGE-1 RevA:3
- Mate:773 (2.3114 mm): Standoff 0.50'':9 ↔ VEX-HINGE-1 RevA:3
- Mate:774: 5 x 30:1 ↔ Standoff 0.50'':10
- Mate:775 (2.3114 mm): 5 x 30:1 ↔ Standoff 0.50'':10
- Mate:776 (2.3114 mm): 5 x 30:1 ↔ Standoff 0.50'':10
- Mate:777 (2.3114 mm): Standoff 0.50'':9 ↔ VEX-HINGE-1 RevA:3
- Mate:778 (2.3114 mm): 5 x 30:1 ↔ Standoff 0.50'':9
- Mate:779: 5 x 30:1 ↔ Standoff 0.50'':9
- Mate:780 (2.3114 mm): 5 x 30:1 ↔ Standoff 0.50'':9
- Flush:63: VEX-HINGE-1 RevA:4 ↔ VEX-HINGE-PIN:4
- Mate:781: VEX-HINGE-1 RevA:4 ↔ VEX-HINGE-PIN:4
- Mate:782: Standoff 0.50'':12 ↔ VEX-HINGE-1 RevA:4
- Mate:783 (2.3114 mm): Standoff 0.50'':11 ↔ VEX-HINGE-1 RevA:4
- Mate:784 (2.3114 mm): Standoff 0.50'':11 ↔ VEX-HINGE-1 RevA:4
- Mate:785 (2.3114 mm): Standoff 0.50'':12 ↔ VEX-HINGE-1 RevA:4
- Flush:64: 2 x 15 custom!!!:2 ↔ 2 x 41103 custom:2
- Flush:65: 2 x 15 custom!!!:2 ↔ 2 x 41103 custom:2
- Flush:66: 2 x 41103 custom:1 ↔ 2 x 15 custom!!!:1
- Flush:67: 2 x 41103 custom:1 ↔ 2 x 15 custom!!!:1
- Mate:788 (2.3114 mm): 2 x 12 c chan:4 ↔ Standoff 0.75'':1
- Mate:789 (2.3114 mm): 2 x 12 c chan:4 ↔ Standoff 0.75'':1
- Mate:790: 2 x 12 c chan:4 ↔ Standoff 0.75'':1
- Mate:791 (2.3114 mm): 2 x 12 c chan:4 ↔ Standoff 0.75'':4
- Mate:792 (2.3114 mm): 2 x 12 c chan:4 ↔ Standoff 0.75'':4
- Mate:793: 2 x 12 c chan:4 ↔ Standoff 0.75'':4
- Mate:794 (2.3114 mm): 2 x 12 c chan:3 ↔ Standoff 0.75'':2
- Mate:795 (2.3114 mm): 2 x 12 c chan:3 ↔ Standoff 0.75'':2
- Mate:796: 2 x 12 c chan:3 ↔ Standoff 0.75'':2
- Mate:797 (2.3114 mm): 2 x 12 c chan:3 ↔ Standoff 0.75'':3
- Mate:798 (2.3114 mm): 2 x 12 c chan:3 ↔ Standoff 0.75'':3
- Mate:799: 2 x 12 c chan:3 ↔ Standoff 0.75'':3
- Mate:800: 2 x 20:1 ↔ Standoff 0.75'':3
- Mate:801 (1.524 mm): 2 x 20:1 ↔ Standoff 0.75'':3
- Mate:802 (2.3114 mm): 2 x 20:1 ↔ Standoff 0.75'':3
- Mate:803 (2.3114 mm): 2 x 20:1 ↔ Standoff 0.75'':4
- Mate:804: Screw 8-32 x 0.250''-Silver:9 ↔ Standoff 0.75'':1
- Mate:805: Screw 8-32 x 0.250''-Silver:9 ↔ 2 x 20:1
- Mate:806: Standoff 0.75'':4 ↔ Screw 8-32 x 0.250''-Silver:10
- Mate:807: 2 x 20:1 ↔ Screw 8-32 x 0.250''-Silver:10
- Mate:808: Standoff 0.75'':3 ↔ Screw 8-32 x 0.250''-Silver:11
- Mate:809: Standoff 0.75'':2 ↔ Screw 8-32 x 0.250''-Silver:12
- Mate:810: 2 x 20:1 ↔ Screw 8-32 x 0.250''-Silver:12
- Mate:811: 2 x 20:1 ↔ Screw 8-32 x 0.250''-Silver:11
- Mate:812: Standoff 0.75'':4 ↔ Screw 8-32 x 0.250''-Silver:13
- Mate:813: Standoff 0.75'':1 ↔ Screw 8-32 x 0.250''-Silver:14
- Mate:814: 2 x 12 c chan:4 ↔ Screw 8-32 x 0.250''-Silver:13
- Mate:815: 2 x 12 c chan:4 ↔ Screw 8-32 x 0.250''-Silver:14
- Mate:818: 1103 laddercustom1:1 ↔ Screw 8-32 x 0.750''-Silver:6
- Mate:819: 1103 laddercustom1:1 ↔ Spacer (Nylon), 0.4375'':1
- Mate:820: Screw 8-32 x 0.750''-Silver:5 ↔ Spacer (Nylon), 0.4375'':2
- Mate:821: 1103 laddercustom1:1 ↔ Spacer (Nylon), 0.4375'':2
- Mate:822: Screw 8-32 x 0.750''-Silver:1 ↔ Spacer (Nylon), 0.4375'':4
- Mate:823: 5 x 30:1 ↔ Spacer (Nylon), 0.4375'':4
- Mate:824: Screw 8-32 x 0.750''-Silver:2 ↔ Spacer (Nylon), 0.4375'':3
- Mate:825: 5 x 30:1 ↔ Spacer (Nylon), 0.4375'':3
- Mate:826: Standoff 0.75'':2 ↔ Screw 8-32 x 0.250''-Silver:16
- Mate:827: Standoff 0.75'':3 ↔ Screw 8-32 x 0.250''-Silver:15
- Mate:828: 2 x 12 c chan:3 ↔ Screw 8-32 x 0.250''-Silver:16
- Mate:829: 2 x 12 c chan:3 ↔ Screw 8-32 x 0.250''-Silver:15
- [Mate]: Standoff 3.00'':1 ↔ Screw 8-32 x 0.500''-Silver:1
- [Mate]: Screw 8-32 x 0.500''-Silver:4 ↔ Standoff 3.00'':2
- Tangent:450: 2 x 12 c chan:2 ↔ .375'' Screw & Nylock Nut (Custom):1
- Tangent:451: 2 x 12 c chan:2 ↔ .375'' Screw & Nylock Nut (Custom):1
- Mate:835: 2 x 12 c chan:2 ↔ .375'' Screw & Nylock Nut (Custom):1
- Tangent:452: 1 x 10:2 ↔ .375'' Screw & Nylock Nut (Custom):1
- Tangent:453: 1 x 10:2 ↔ .375'' Screw & Nylock Nut (Custom):1
- Mate:836: .375'' Screw & Nylock Nut (Custom):1 ↔ .375'' Screw & Nylock Nut (Custom):2
- Mate:837: 2 x 12 c chan:1 ↔ .375'' Screw & Nylock Nut (Custom):2
- Tangent:454: 2 x 12 c chan:2 ↔ .375'' Screw & Nylock Nut:1
- Tangent:455: 2 x 12 c chan:2 ↔ .375'' Screw & Nylock Nut:1
- Mate:838: 2 x 12 c chan:2 ↔ .375'' Screw & Nylock Nut:1
- Tangent:456: 2 x 12 c chan:2 ↔ .375'' Screw & Nylock Nut:4
- Tangent:457: 2 x 12 c chan:2 ↔ .375'' Screw & Nylock Nut:4
- Mate:839: 2 x 12 c chan:2 ↔ .375'' Screw & Nylock Nut:4
- Tangent:458: 2 x 12 c chan:1 ↔ .375'' Screw & Nylock Nut:3
- Tangent:459: 2 x 12 c chan:1 ↔ .375'' Screw & Nylock Nut:3
- Mate:840: 2 x 12 c chan:1 ↔ .375'' Screw & Nylock Nut:3
- Tangent:460: 2 x 12 c chan:1 ↔ .375'' Screw & Nylock Nut:2
- Tangent:461: 2 x 12 c chan:1 ↔ .375'' Screw & Nylock Nut:2
- Mate:841: 2 x 12 c chan:1 ↔ .375'' Screw & Nylock Nut:2
- Tangent:462: 2 x 12 c chan:3 ↔ .375'' Screw & Nylock Nut:1
- Tangent:463: 2 x 12 c chan:3 ↔ .375'' Screw & Nylock Nut:1
- Mate:843: 1 x 10:1 ↔ .375'' Screw & Nylock Nut:5
- Mate:845: 1 x 10:2 ↔ .375'' Screw & Nylock Nut:6
- Mate:846: Standoff 0.50'':6 ↔ Screw 8-32 x 0.250''-Silver:20
- Mate:847: VEX-HINGE-1 RevA:1 ↔ Screw 8-32 x 0.250''-Silver:20
- Mate:848: Standoff 0.50'':8 ↔ Screw 8-32 x 0.250''-Silver:17
- Mate:849: VEX-HINGE-1 RevA:1 ↔ Screw 8-32 x 0.250''-Silver:17
- Mate:850: Standoff 0.50'':11 ↔ Screw 8-32 x 0.250''-Silver:18
- Mate:851: VEX-HINGE-1 RevA:4 ↔ Screw 8-32 x 0.250''-Silver:18
- Mate:852: Standoff 0.50'':12 ↔ Screw 8-32 x 0.250''-Silver:19
- Mate:853: VEX-HINGE-1 RevA:4 ↔ Screw 8-32 x 0.250''-Silver:19
- Mate:854: Standoff 0.50'':5 ↔ Screw 8-32 x 0.250''-Silver:21
- Mate:855: VEX-HINGE-1 RevA:2 ↔ Screw 8-32 x 0.250''-Silver:21
- Mate:856: Standoff 0.50'':7 ↔ Screw 8-32 x 0.250''-Silver:22
- Mate:857: VEX-HINGE-1 RevA:2 ↔ Screw 8-32 x 0.250''-Silver:22
- Mate:858: Standoff 0.50'':10 ↔ Screw 8-32 x 0.250''-Silver:23
- Mate:859: VEX-HINGE-1 RevA:3 ↔ Screw 8-32 x 0.250''-Silver:23
- Mate:860: Standoff 0.50'':9 ↔ Screw 8-32 x 0.250''-Silver:24
- Mate:861: VEX-HINGE-1 RevA:3 ↔ Screw 8-32 x 0.250''-Silver:24
- [Mate] (2.3114 mm): 5 x 30:1 ↔ Screw 8-32 x 0.875''-Silver:1
- [Mate] (2.3114 mm): 5 x 30:1 ↔ Screw 8-32 x 0.875''-Silver:1
- [Mate]: 5 x 30:1 ↔ Screw 8-32 x 0.875''-Silver:1
- Mate:865: Screw 8-32 x 0.875''-Silver:1 ↔ Nut 8-32 Nylock:21
- [Mate]: Screw 8-32 x 0.875''-Silver:1 ↔ Spacer (Nylon), 0.375'':7
- [Mate]: 5 x 30:1 ↔ Spacer (Nylon), 0.375'':7
- Mate:868 (3.048 mm): Spacer (Nylon), 0.375'':7 ↔ High Strength Chain Link:1
- Mate:869 (6.096 mm): Nut 8-32 Nylock:21 ↔ Spacer (Nylon), 0.375'':7
- Tangent:466: Screw 8-32 x 0.875''-Silver:1 ↔ High Strength Chain Link:1
- Mate:870 (3.048 mm): Spacer (Nylon), 0.375'':7 ↔ High Strength Chain Link:1
- Tangent:467 (1.8542 mm): Screw 8-32 x 0.875''-Silver:1 ↔ High Strength Chain Link:1
- Mate:871: High Strength Chain Link:1 ↔ High Strength Chain Link:2
- Flush:68: High Strength Chain Link:1 ↔ High Strength Chain Link:2
- Mate:872: 1 x 10:1 ↔ Screw 8-32 x 0.500''-Silver:2
- Mate:873 (-1.27 mm): Spacer (Nylon), 0.250'':1 ↔ Standoff 3.00'':2
- Mate:874 (-1.27 mm): Spacer (Nylon), 0.250'':3 ↔ Standoff 3.00'':2
- Mate:875: 2 x 12 c chan:4 ↔ 1 x 10:1
- Mate:876 (4.6228 mm): 2 x 12 c chan:3 ↔ .375'' Screw & Nylock Nut:6
- Mate:877: 2 x 12 c chan:3 ↔ .375'' Screw & Nylock Nut:6
- Tangent:468: 1 x 10:2 ↔ .375'' Screw & Nylock Nut:6
- Tangent:469: 1 x 10:2 ↔ .375'' Screw & Nylock Nut:6
- Mate:878: .375'' Screw & Nylock Nut:5 ↔ .375'' Screw & Nylock Nut:6
- Mate:879: Screw 8-32 x 0.625''-Silver:2 ↔ Ladder Mech:1
- Mate:880: Screw 8-32 x 0.625''-Silver:1 ↔ Ladder Mech:1
- Mate:881 (18.796 mm): 2 x 12 c chan:4 ↔ Ladder Mech:1
- Mate:882: Ladder Mech:1 ↔ Screw 8-32 x 0.750''-Silver:7
- Mate:883: Ladder Mech:1 ↔ Screw 8-32 x 0.750''-Silver:8
- Mate:884: 2 x 12 c chan:4 ↔ Screw 8-32 x 0.750''-Silver:8
- Mate:885: 2 x 12 c chan:3 ↔ Screw 8-32 x 0.750''-Silver:7
- Mate:886: Screw 8-32 x 0.625''-Silver:1 ↔ Nut 8-32 Nylock:25
- Mate:887: Screw 8-32 x 0.750''-Silver:7 ↔ Nut 8-32 Nylock:24
- Mate:888: Screw 8-32 x 0.750''-Silver:8 ↔ Nut 8-32 Nylock:22
- Mate:889: Screw 8-32 x 0.625''-Silver:2 ↔ Nut 8-32 Nylock:23
- Angle:1 (65 deg): 2 x 12 c chan:2 ↔ Ladder Mech:1
- Mate:890 (-7.874 mm): Screw 8-32 x 0.625''-Silver:2 ↔ Nut 8-32 Nylock:23
- Mate:891 (-8.128 mm): Screw 8-32 x 0.625''-Silver:1 ↔ Nut 8-32 Nylock:25
- Mate:892 (-5.588 mm): Screw 8-32 x 0.750''-Silver:7 ↔ Nut 8-32 Nylock:24
- Mate:893 (-5.588 mm): Screw 8-32 x 0.750''-Silver:8 ↔ Nut 8-32 Nylock:22
- Mate:894: 2 x 15 custom!!!:1 ↔ Screw 8-32 x 1.250''-Silver:1
- Mate:895: Nut 8-32 Nylock:26 ↔ Screw 8-32 x 1.250''-Silver:1
- Mate:896: 2 x 15 custom!!!:1 ↔ Nut 8-32 Nylock:26
- Mate:897: 2 x 15 custom!!!:1 ↔ Screw 8-32 x 1.250''-Silver:1
- Mate:898: 2 x 15 custom!!!:2 ↔ Screw 8-32 x 1.250''-Silver:2
- Mate:900: 2 x 15 custom!!!:2 ↔ Nut 8-32 Nylock:27
- Mate:901: 2 x 15 custom!!!:2 ↔ Screw 8-32 x 1.250''-Silver:2
- Mate:902: Nut 8-32 Nylock:27 ↔ Screw 8-32 x 1.250''-Silver:2
- Mate:903: 2 x 15 custom!!!:2 ↔ 2 x 41103 custom:2
- Mate:904: 2 x 41103 custom:1 ↔ 2 x 15 custom!!!:1
- Mate:905: Standoff 0.50'':6 ↔ VEX-HINGE-1 RevA:1
